# Autodesk Inventor assembly: pulleyassebly
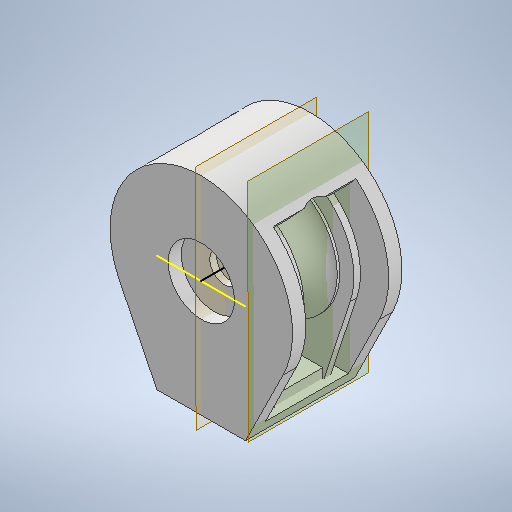
[picture p0: Inventor's stored thumbnail of the model, 512x512]
Saved by Autodesk Inventor 2025.2 (Build 292293000, 293)
## iProperties
Created: 2025-01-13
Part Number: pulleyassebly
Document SubType Name: Assembly
Designer: email
Author: email
## Documents named in this file (4)
- C:\Users\email\Desktop\Projects\Capstone\4TB6\CAD_Model\thigh_mount\pulleyassebly.iam
- C:\Users\email\Desktop\Projects\Capstone\4TB6\CAD_Model\pidtest\pulley.ipt
- C:\Users\email\Desktop\Projects\Capstone\4TB6\CAD_Model\pidtest\pulleybearing.ipt
- C:\Users\email\Desktop\Projects\Capstone\4TB6\CAD_Model\thigh_mount\pulleyblocker.ipt
## Components (3 placed, 3 different names)
1. pulley:1 — Mate:1, Mate:2, Mate:3, Mate:4
2. pulleybearing:1 — Mate:1, Mate:2
3. pulleyblocker:1 — Mate:3, Mate:4
## Relationships (4: Mate 4)
- Mate:1: pulley:1 ↔ pulleybearing:1
- Mate:2 (1 mm): pulley:1 ↔ pulleybearing:1
- Mate:3: pulley:1 ↔ pulleyblocker:1
- Mate:4 (3 mm): pulley:1 ↔ pulleyblocker:1
